# Autodesk Inventor assembly: Drive Gear Assembly
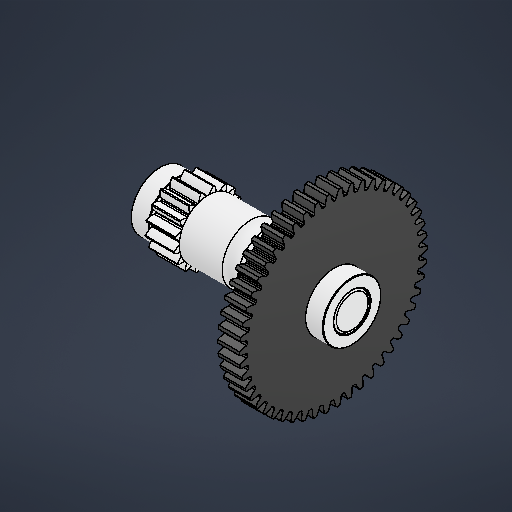
[picture p0: Inventor's stored thumbnail of the model, 512x512]
Saved by Autodesk Inventor 2026 (Build 300175050, 175E)
## iProperties
Created: 2025-05-11
Part Number: Drive Gear Assembly
Document SubType Name: Assembly
Designer: Joshua Eah
Author: Joshua Eah
## Documents named in this file (4)
- C:\Users\Joshua Eah\Documents\GitHub\Voron-0\CAD\Master Assembly\Toolhead\Subassemblies\Drive Gear Assembly.iam
- C:\Users\Joshua Eah\Documents\GitHub\Voron-0\CAD\Master Assembly\Toolhead\Parts\Extruder\MR85 Bearing.ipt
- C:\Users\Joshua Eah\Documents\GitHub\Voron-0\CAD\Master Assembly\Toolhead\Parts\Extruder\Drive Gear.ipt
- C:\Users\Joshua Eah\Documents\GitHub\Voron-0\CAD\Master Assembly\Toolhead\Parts\Extruder\50 Tooth Gear.ipt
## Components (4 placed, 3 different names)
1. MR85 Bearing:1 — Insert:2
2. Drive Gear:1 — Insert:3
3. 50 Tooth Gear:1 — Insert:1, Insert:2
4. MR85 Bearing:2 — Insert:1, Insert:3
## Relationships (3: Insert 3)
- Insert:1: 50 Tooth Gear:1 ↔ MR85 Bearing:2
- Insert:2: MR85 Bearing:1 ↔ 50 Tooth Gear:1
- Insert:3 (0.2 mm): Drive Gear:1 ↔ MR85 Bearing:2
